# Autodesk Inventor assembly: stepper_28
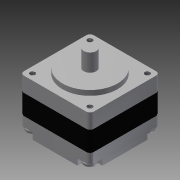
[picture p0: Inventor's stored thumbnail of the model, 180x180]
Saved by Autodesk Inventor 2013 (Build 170138000, 138)
## iProperties
Shininess: 20.0
Created: 2013-02-12
Part Number: stepper_28
Document SubType Name: Assembly
Designer: Noa Izumi
Density: 0.0
Volumn: 0.0
Area: 0.0
PropertySet Name: Model Information
Control State: 0
Master: False
Checked Out: False
Author: Noa Izumi
## Documents named in this file (5)
- C:\reprap\reprap_13\stepper_28.iam
- C:\reprap\reprap_13\stepper_front_28.ipt
- C:\reprap\reprap_13\stepper_middle_28.ipt
- C:\reprap\reprap_13\stepper_bottom_28.ipt
- C:\reprap\reprap_13\screw_M3_5.ipt
## Components (7 placed, 4 different names)
1. stepper_front_28:1 — 插入:1, 插入:2
2. stepper_middle_28:1 — 插入:1, 插入:2, 插入:3, 插入:4
3. stepper_bottom_28:1 — 插入:3, 插入:4, 插入:5, 插入:6, 插入:7, 插入:8
4. screw_M3_5:1 — 插入:5
5. screw_M3_5:2 — 插入:6
6. screw_M3_5:3 — 插入:7
7. screw_M3_5:4 — 插入:8
## Relationships (8: Insert 8)
- 插入:1 [Insert]: stepper_front_28:1 ↔ stepper_middle_28:1
- 插入:2 [Insert]: stepper_front_28:1 ↔ stepper_middle_28:1
- 插入:3 [Insert]: stepper_middle_28:1 ↔ stepper_bottom_28:1
- 插入:4 [Insert]: stepper_middle_28:1 ↔ stepper_bottom_28:1
- 插入:5 [Insert]: stepper_bottom_28:1 ↔ screw_M3_5:1
- 插入:6 [Insert]: stepper_bottom_28:1 ↔ screw_M3_5:2
- 插入:7 [Insert]: stepper_bottom_28:1 ↔ screw_M3_5:3
- 插入:8 [Insert]: stepper_bottom_28:1 ↔ screw_M3_5:4
